# Autodesk Inventor assembly: osszeallitas
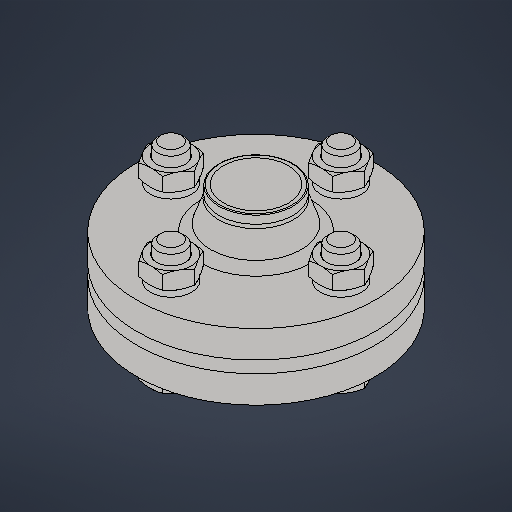
[picture p0: Inventor's stored thumbnail of the model, 512x512]
Saved by Autodesk Inventor 2026.1 (Build 301233020, 233B)
## iProperties
Created: 2025-10-06
Part Number: osszeallitas
Document SubType Name: Assembly
Designer: Agi
Author: Agi
## Documents named in this file (7)
- C:\Users\User\Documents\GitHub\Gepelemek1HF\Inventor\osszeallitas.iam
- C:\Users\User\Documents\GitHub\Gepelemek1HF\Inventor\csavar.ipt
- C:\Users\User\Documents\GitHub\Gepelemek1HF\Inventor\csavaranya.ipt
- C:\Users\User\Documents\GitHub\Gepelemek1HF\Inventor\karima.ipt
- C:\Users\User\Documents\GitHub\Gepelemek1HF\Inventor\tomites.ipt
- C:\Users\User\Documents\GitHub\Gepelemek1HF\Inventor\vakkarima.ipt
- C:\Users\User\Documents\GitHub\Gepelemek1HF\Inventor\alatet.ipt
## Components (15 placed, 6 different names)
1. karima:1 — Mate:1, Mate:2, Mate:3, Mate:4, Mate:6, Mate:11
2. tomites:1 — Mate:1, Mate:2, Mate:3, Mate:5
3. vakkarima:1 — Mate:4, Mate:5, Mate:6, Mate:7, Mate:8, Mate:9
4. csavaranya:1 — Mate:12, Mate:13, Flush:1
5. alatet:1 — Mate:10, Mate:11, Mate:13, Mate:14
6. csavar:1 — Mate:7, Mate:8, Mate:9, Mate:10, Mate:12, Flush:1, Mate:14
7. csavaranya:2
8. alatet:2
9. csavar:2
10. csavaranya:3
11. alatet:3
12. csavar:3
13. csavaranya:4
14. alatet:4
15. csavar:4
## Component patterns: (4 elements, first: csavaranya:1 + alatet:1 + csavar:1)
## Relationships (15: Mate 14, Flush 1)
- Mate:1: karima:1 ↔ tomites:1
- Mate:2: karima:1 ↔ tomites:1
- Mate:3: karima:1 ↔ tomites:1
- Mate:4: karima:1 ↔ vakkarima:1
- Mate:5: tomites:1 ↔ vakkarima:1
- Mate:6: karima:1 ↔ vakkarima:1
- Mate:7: vakkarima:1 ↔ csavar:1
- Mate:8: vakkarima:1 ↔ csavar:1
- Mate:9: vakkarima:1 ↔ csavar:1
- Mate:10: alatet:1 ↔ csavar:1
- Mate:11: karima:1 ↔ alatet:1
- Mate:12: csavaranya:1 ↔ csavar:1
- Mate:13: csavaranya:1 ↔ alatet:1
- Flush:1: csavaranya:1 ↔ csavar:1
- Mate:14: alatet:1 ↔ csavar:1
